# Autodesk Inventor assembly: TeaTime
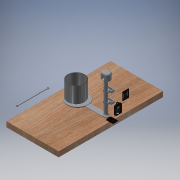
[picture p0: Inventor's stored thumbnail of the model, 180x180]
Saved by Autodesk Inventor 2019 (Build 230136000, 136)
## iProperties
Created: 2020-10-30
Part Number: TeaTime
Document SubType Name: Assembly
Designer: Mike
Author: Mike
## Documents named in this file (10)
- G:\My Drive\Projects\TeaTime\TeaTime.iam
- G:\My Drive\Projects\TeaTime\Mug.ipt
- G:\My Drive\Projects\TeaTime\Table.ipt
- G:\My Drive\Projects\PiCanon\Downloads\raspberry-pi-27.snapshot.7\WEMOS-D1-mini_stl.ipt
- G:\My Drive\Projects\TeaTime\base2.ipt
- G:\My Drive\Projects\TeaTime\fishing_rod.ipt
- G:\My Drive\Projects\TeaTime\top.ipt
- G:\My Drive\Projects\PiCanon\Downloads\raspberry-pi-27.snapshot.7\Mini_Keychain_Base_Logo.ipt
- G:\My Drive\Projects\PiCanon\Downloads\raspberry-pi-27.snapshot.7\Mini_Keychain_Cap_Logo.ipt
- G:\My Drive\Projects\TeaTime\clip.ipt
## Components (10 placed, 9 different names)
1. Mug:1 — Mate:3
2. Table:1 — Mate:1, Mate:2, Flush:1, Mate:3, Mate:4
3. WEMOS-D1-mini_stl:1
4. base2:1 — Mate:4, Mate:5, Mate:6, Mate:7
5. fishing_rod:1
6. top:1 — Mate:5
7. Mini_Keychain_Base_Logo:1
8. Mini_Keychain_Cap_Logo:1
9. clip:1 — Mate:6
10. clip:2 — Mate:7
## Relationships (8: Mate 7, Flush 1)
- Mate:1: Table:1
- Mate:2: Table:1
- Flush:1: Table:1
- Mate:3: Mug:1 ↔ Table:1
- Mate:4: Table:1 ↔ base2:1
- Mate:5: base2:1 ↔ top:1
- Mate:6: base2:1 ↔ clip:1
- Mate:7: base2:1 ↔ clip:2
